# Autodesk Inventor assembly: Корпус электроники
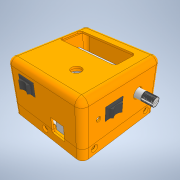
[picture p0: Inventor's stored thumbnail of the model, 180x180]
Saved by Autodesk Inventor 2021.1 (Build 251245010, 245A)
## iProperties
Created: 2026-06-28
Part Number: Корпус электроники
Document SubType Name: Assembly
Designer: Андрей Тарасов
Author: Андрей Тарасов
## Documents named in this file (6)
- G:\04. Inventor\024. EDM 3.0\Корпус электроники.iam
- G:\04. Inventor\024. EDM 3.0\Дно корпуса электроники.ipt
- G:\04. Inventor\024. EDM 3.0\Плата.ipt
- G:\04. Inventor\024. EDM 3.0\Крышка корпуса электроники.ipt
- G:\04. Inventor\024. EDM 3.0\Выключатель маленький.ipt
- G:\04. Inventor\024. EDM 3.0\Потенциометр маленький.ipt
## Components (6 placed, 5 different names)
1. Плата:1 — Совмещение:16, Совмещение:17, Совмещение:18
2. Крышка корпуса электроники:1 — Совмещение:4, Заподлицо:1, Заподлицо:2, Совмещение:8, Совмещение:9, Совмещение:10, Совмещение:11, Совмещение:12, Совмещение:13, Совмещение:14, Совмещение:15
3. Дно корпуса электроники:1 — Совмещение:4, Заподлицо:1, Заподлицо:2, Совмещение:16, Совмещение:17, Совмещение:18
4. Выключатель маленький:1 — Совмещение:9, Совмещение:10, Совмещение:11
5. Выключатель маленький:2 — Совмещение:13, Совмещение:14, Совмещение:15
6. Потенциометр маленький:1 — Совмещение:8, Совмещение:12
## Relationships (14: Mate 12, Flush 2)
- Совмещение:4 [Mate]: Крышка корпуса электроники:1 ↔ Дно корпуса электроники:1
- Заподлицо:1 [Flush]: Крышка корпуса электроники:1 ↔ Дно корпуса электроники:1
- Заподлицо:2 [Flush]: Крышка корпуса электроники:1 ↔ Дно корпуса электроники:1
- Совмещение:8 [Mate]: Крышка корпуса электроники:1 ↔ Потенциометр маленький:1
- Совмещение:9 [Mate]: Крышка корпуса электроники:1 ↔ Выключатель маленький:1
- Совмещение:10 [Mate]: Крышка корпуса электроники:1 ↔ Выключатель маленький:1
- Совмещение:11 [Mate]: Крышка корпуса электроники:1 ↔ Выключатель маленький:1
- Совмещение:12 [Mate]: Крышка корпуса электроники:1 ↔ Потенциометр маленький:1
- Совмещение:13 [Mate]: Крышка корпуса электроники:1 ↔ Выключатель маленький:2
- Совмещение:14 [Mate]: Крышка корпуса электроники:1 ↔ Выключатель маленький:2
- Совмещение:15 [Mate]: Крышка корпуса электроники:1 ↔ Выключатель маленький:2
- Совмещение:16 [Mate]: Плата:1 ↔ Дно корпуса электроники:1
- Совмещение:17 [Mate]: Плата:1 ↔ Дно корпуса электроники:1
- Совмещение:18 [Mate]: Плата:1 ↔ Дно корпуса электроники:1
